# Autodesk Inventor assembly: Устройство сопряжения
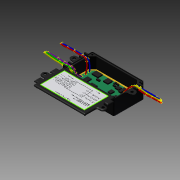
[picture p0: Inventor's stored thumbnail of the model, 180x180]
Saved by Autodesk Inventor 2012 (Build 160160000, 160)
## iProperties
Created: 2009-09-08
Part Number: Устройство сопряжения
Document SubType Name: Assembly
Designer: toma
Mass: 20.407 g
Surface Area: 285.289 cm^2
Volume: 20.407 cm^3
Density: 1 g/cm^3
Author: toma
## Documents named in this file (10)
- D:\VSS_WORK\VSS_ENERGO\Устройство сопряжения ДУТ 3.0 light\КД\УС ДУТ light частотный\Устройство сопряжения.iam
- D:\VSS_WORK\VSS_ENERGO\Устройство сопряжения ДУТ 3.0 light\КД\УС ДУТ light частотный\корпус.ipt
- D:\VSS_WORK\VSS_ENERGO\Устройство сопряжения ДУТ 3.0 light\КД\УС ДУТ light частотный\Сборка платы.iam
- D:\VSS_WORK\VSS_ENERGO\Устройство сопряжения ДУТ 3.0 light\КД\УС ДУТ light частотный\клей.ipt
- D:\VSS_WORK\VSS_ENERGO\Устройство сопряжения ДУТ 3.0 light\КД\УС ДУТ light частотный\контакт.ipt
- D:\Inventor\рабочая папка\Устройство сопряжения\Устройство сопряжения.Прокладка кабелей1.iam
- D:\Inventor\рабочая папка\Устройство сопряжения\Устройство сопряжения.Прокладка кабелей2.iam
- D:\Inventor\рабочая папка\Устройство сопряжения\Устройство сопряжения.Прокладка кабелей3.iam
- D:\Inventor\рабочая папка\Устройство сопряжения\Устройство сопряжения.Прокладка кабелей4.iam
- D:\VSS_WORK\VSS_ENERGO\Устройство сопряжения ДУТ 3.0 light\КД\УС ДУТ light частотный\Сборка1.iam
## Components (16 placed, 9 different names)
1. корпус:1 — Совмещение:1, Совмещение:2, Совмещение:3, Совмещение:6, Совмещение:7, Совмещение:8, Совмещение:10, Совмещение:11, Совмещение:12, Совмещение:13, Совмещение:14, Совмещение:15, Совмещение:16, Совмещение:17, Совмещение:18, Совмещение:19, Совмещение:20, Совмещение:21, Совмещение:22, Совмещение:23, Совмещение:24, Совмещение:25, Совмещение:26, Совмещение:27, Совмещение:28, Совмещение:29, Совмещение:30, Совмещение:31, Совмещение:32, Совмещение:33
2. Сборка платы:1 [sub-assembly] — Совмещение:1, Совмещение:2, Совмещение:3, Совмещение:4, Совмещение:5
3. клей:1 — Совмещение:4, Совмещение:5
4. контакт:1 — Совмещение:6, Совмещение:7, Совмещение:8
5. Прокладка кабелей1 [sub-assembly]
6. контакт:2 — Совмещение:10, Совмещение:11, Совмещение:12
7. контакт:3 — Совмещение:13, Совмещение:14, Совмещение:15
8. Прокладка кабелей2 [sub-assembly]
9. Прокладка кабелей3 [sub-assembly]
10. контакт:4 — Совмещение:16, Совмещение:17, Совмещение:18
11. контакт:5 — Совмещение:19, Совмещение:20, Совмещение:21
12. контакт:6 — Совмещение:22, Совмещение:23, Совмещение:24
13. контакт:7 — Совмещение:25, Совмещение:26, Совмещение:27
14. контакт:8 — Совмещение:28, Совмещение:29, Совмещение:30
15. Прокладка кабелей4 [sub-assembly]
16. Сборка1:1 [sub-assembly] — Совмещение:31, Совмещение:32, Совмещение:33
## Relationships (32: Mate 32)
- Совмещение:1 [Mate] (2 mm): корпус:1 ↔ Сборка платы:1
- Совмещение:2 [Mate] (1.5 mm): корпус:1 ↔ Сборка платы:1
- Совмещение:3 [Mate] (2 mm): корпус:1 ↔ Сборка платы:1
- Совмещение:4 [Mate]: Сборка платы:1 ↔ клей:1
- Совмещение:5 [Mate]: Сборка платы:1 ↔ клей:1
- Совмещение:6 [Mate] (1.2 mm): корпус:1 ↔ контакт:1
- Совмещение:7 [Mate] (0.5 mm): корпус:1 ↔ контакт:1
- Совмещение:8 [Mate] (28 mm): корпус:1 ↔ контакт:1
- Совмещение:10 [Mate] (30 mm): корпус:1 ↔ контакт:2
- Совмещение:11 [Mate] (2.5 mm): корпус:1 ↔ контакт:2
- Совмещение:12 [Mate] (1.5 mm): корпус:1 ↔ контакт:2
- Совмещение:13 [Mate] (28 mm): корпус:1 ↔ контакт:3
- Совмещение:14 [Mate] (1.2 mm): корпус:1 ↔ контакт:3
- Совмещение:15 [Mate] (0.5 mm): корпус:1 ↔ контакт:3
- Совмещение:16 [Mate] (30 mm): корпус:1 ↔ контакт:4
- Совмещение:17 [Mate] (1.5 mm): корпус:1 ↔ контакт:4
- Совмещение:18 [Mate] (1.5 mm): корпус:1 ↔ контакт:4
- Совмещение:19 [Mate] (3.3 mm): корпус:1 ↔ контакт:5
- Совмещение:20 [Mate] (1.3 mm): корпус:1 ↔ контакт:5
- Совмещение:21 [Mate] (30 mm): корпус:1 ↔ контакт:5
- Совмещение:22 [Mate] (29 mm): корпус:1 ↔ контакт:6
- Совмещение:23 [Mate] (4.8 mm): корпус:1 ↔ контакт:6
- Совмещение:24 [Mate] (0.6 mm): корпус:1 ↔ контакт:6
- Совмещение:25 [Mate] (30 mm): корпус:1 ↔ контакт:7
- Совмещение:26 [Mate] (2 mm): корпус:1 ↔ контакт:7
- Совмещение:27 [Mate] (0.7 mm): корпус:1 ↔ контакт:7
- Совмещение:28 [Mate] (30 mm): корпус:1 ↔ контакт:8
- Совмещение:29 [Mate] (3.5 mm): корпус:1 ↔ контакт:8
- Совмещение:30 [Mate] (0.8 mm): корпус:1 ↔ контакт:8
- Совмещение:31 [Mate]: корпус:1 ↔ Сборка1:1
- Совмещение:32 [Mate] (1 mm): корпус:1 ↔ Сборка1:1
- Совмещение:33 [Mate] (2 mm): корпус:1 ↔ Сборка1:1
